# Autodesk Inventor assembly: Lower_Arm_ConnectorJe19
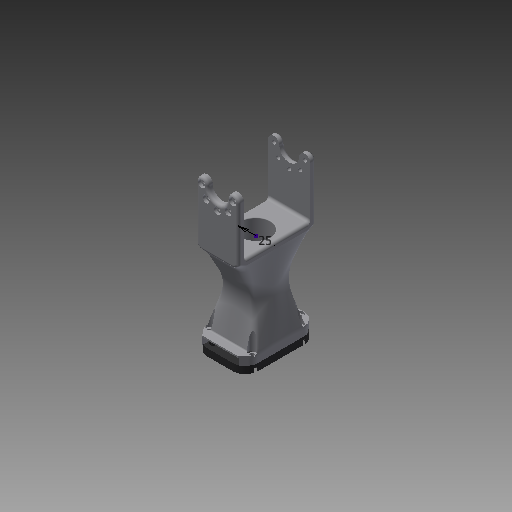
[picture p0: Inventor's stored thumbnail of the model, 512x512]
Saved by Autodesk Inventor 2019 (Build 230136000, 136)
## iProperties
Created: 2019-06-24
Part Number: Lower_Arm_ConnectorJe19
Document SubType Name: Assembly
Designer: xwermter
Author: xwermter
## Documents named in this file (3)
- Z:\Nico_N\NICO-CAD-master\NICO_CAD_master\arms\Lower_Arm_ConnectorJe19.iam
- Z:\NICO_CAD\NICO-CAD\NICO_CAD_master\arms\arms\lower_arm_thick1.ipt
- Z:\NICO_CAD\NICO-CAD\Nico_CAD_N\Nico_N\NICO-CAD-master\NICO_CAD_master\arms\arms\connector.ipt
## Components (2 placed, 2 different names)
1. lower_arm_thick1:1 — Mate:1, Mate:2
2. connector:1 — Mate:1, Mate:2
## Relationships (2: Mate 2)
- Mate:1: lower_arm_thick1:1 ↔ connector:1
- Mate:2: lower_arm_thick1:1 ↔ connector:1
